# Autodesk Inventor assembly: Arm1.2ProtoAssembly
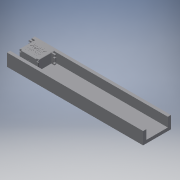
[picture p0: Inventor's stored thumbnail of the model, 180x180]
Saved by Autodesk Inventor 2017 (Build 210142000, 142)
## iProperties
Created: 2017-09-30
Part Number: Arm1.2ProtoAssembly
Document SubType Name: Assembly
Designer: User
Author: User
## Documents named in this file (3)
- C:\Robotics\CAD\2017-18_CAD\Arm1.2ProtoAssembly.iam
- C:\Robotics\CAD\2017-18_CAD\ArmProto1.2.ipt
- C:\Robotics\CAD\COTSParts\Vex\REV-41-1097.iam
## Components (2 placed, 2 different names)
1. ArmProto1.2:1 — Flush:1, Flush:2, Mate:1
2. REV-41-1097:1 [sub-assembly] — Flush:1, Flush:2, Mate:1
## Relationships (3: Flush 2, Mate 1)
- Flush:1: ArmProto1.2:1 ↔ REV-41-1097:1
- Flush:2: ArmProto1.2:1 ↔ REV-41-1097:1
- Mate:1: ArmProto1.2:1 ↔ REV-41-1097:1
